# Autodesk Inventor assembly: Assembly1
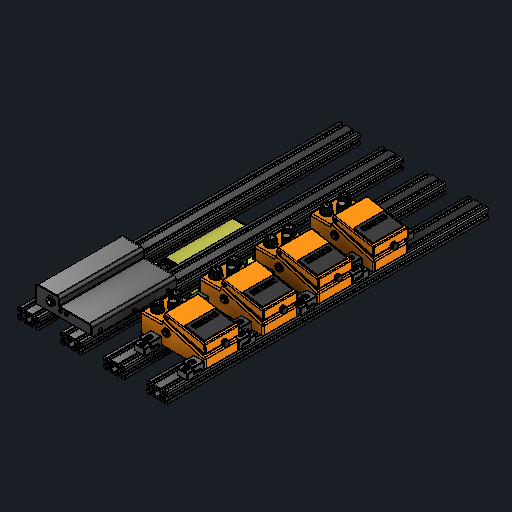
[picture p0: Inventor's stored thumbnail of the model, 512x512]
Saved by Autodesk Inventor 2026.2 (Build 302298000, 298)
## iProperties
Created: 2026-07-17
Part Number: Assembly1
Document SubType Name: Assembly
Designer: JoshuaEah
Author: JoshuaEah
## Documents named in this file (7)
- C:\Users\JoshuaEah\Documents\GitHub\Designed-Trinkets\Guitar\Modular Pedalboard\Assembly1.iam
- C:\Users\JoshuaEah\Documents\GitHub\Designed-Trinkets\Guitar\Modular Pedalboard\Pedals\Boss Pedal\Boss_Assembly.iam
- C:\Users\JoshuaEah\Documents\GitHub\Designed-Trinkets\Guitar\Modular Pedalboard\Fixtures\Fixture Assembly (M4).iam
- C:\Users\JoshuaEah\Documents\GitHub\Designed-Trinkets\Guitar\Modular Pedalboard\Pedals\SuperBlock US\SuperBlock US.iam
- C:\Users\JoshuaEah\Documents\GitHub\Designed-Trinkets\Guitar\Modular Pedalboard\Pedals\Power Supply\VITOOS AD5S LINK.iam
- C:\Users\JoshuaEah\Documents\GitHub\Designed-Trinkets\Guitar\Modular Pedalboard\Hardware\2040x60cm Extrusion.ipt
- 2040x60cm Extrusion.ipt
## Components (26 placed, 5 different names)
1. 2040x60cm Extrusion:5 — Mate:1, Rigid:1, Mate:2, Mate:3, Angle:1, Flush:1, Rigid:2, Mate:6, Mate:8, Planar:1, Flush:4, Flush:5, Planar:6, Planar:7, Mate:18, Mate:19, Mate:29, Mate:30, Planar:9, Flush:6, Planar:11, Mate:38, Mate:40, Planar:15, Planar:16, Flush:7
2. 2040x60cm Extrusion:6 — Rigid:1, Mate:11, Planar:2, Planar:3, Mate:12, Planar:4, Planar:5, Mate:14, Mate:15, Mate:26, Mate:27, Mate:28, Planar:8, Planar:10, Mate:37, Mate:39, Mate:41, Planar:13, Planar:14
3. 2040x60cm Extrusion:7 — Rigid:2, Rigid:3, Mate:31, Mate:32, Planar:12
4. 2040x60cm Extrusion:8 — Rigid:3
5. Boss_Assembly:1 [sub-assembly] — Mate:2, Mate:9, Mate:10, Mate:13, Flush:5, Mate:42
6. Fixture Assembly (M4):1 [sub-assembly] — Mate:3, Angle:1, Flush:1, Mate:10
7. Fixture Assembly (M4):2 [sub-assembly] — Mate:8, Planar:1, Mate:9
8. Fixture Assembly (M4):3 [sub-assembly] — Mate:11, Planar:2, Mate:42
9. Fixture Assembly (M4):4 [sub-assembly] — Planar:3, Mate:12, Mate:13
10. Boss_Assembly:2 [sub-assembly] — Mate:6, Mate:16, Mate:17, Flush:4, Mate:20, Mate:21
11. Fixture Assembly (M4):5 [sub-assembly] — Planar:4, Mate:14, Mate:16
12. Fixture Assembly (M4):6 [sub-assembly] — Planar:5, Mate:15, Mate:17
13. Fixture Assembly (M4):7 [sub-assembly] — Planar:6, Mate:18, Mate:20
14. Fixture Assembly (M4):8 [sub-assembly] — Planar:7, Mate:19, Mate:21
15. Boss_Assembly:3 [sub-assembly] — Mate:25, Mate:27, Flush:6
16. Fixture Assembly (M4):9 [sub-assembly] — Mate:29, Planar:11
17. Fixture Assembly (M4):10 [sub-assembly] — Mate:30, Planar:9
18. Fixture Assembly (M4):11 [sub-assembly] — Mate:25, Mate:26, Planar:8
19. Fixture Assembly (M4):12 [sub-assembly] — Mate:28, Planar:10
20. Boss_Assembly:4 [sub-assembly] — Mate:41, Flush:7
21. Fixture Assembly (M4):13 [sub-assembly] — Mate:37, Planar:13
22. Fixture Assembly (M4):14 [sub-assembly] — Mate:39, Planar:14
23. Fixture Assembly (M4):15 [sub-assembly] — Mate:38, Planar:16
24. Fixture Assembly (M4):16 [sub-assembly] — Mate:40, Planar:15
25. SuperBlock US:1 [sub-assembly] — Mate:31
26. VITOOS AD5S LINK:1 [sub-assembly] — Mate:32, Planar:12
## Relationships (64: Mate 39, PlanarJoint 16, Flush 5, WeldJoint 3, Angle 1)
- Mate:1: 2040x60cm Extrusion:5
- Rigid:1 [WeldJoint] (40 mm): 2040x60cm Extrusion:5 ↔ 2040x60cm Extrusion:6
- Mate:2: 2040x60cm Extrusion:5 ↔ Boss_Assembly:1
- Mate:3: 2040x60cm Extrusion:5 ↔ Fixture Assembly (M4):1
- Angle:1 (0 deg): 2040x60cm Extrusion:5 ↔ Fixture Assembly (M4):1
- Flush:1: 2040x60cm Extrusion:5 ↔ Fixture Assembly (M4):1
- Rigid:2 [WeldJoint] (40 mm): 2040x60cm Extrusion:5 ↔ 2040x60cm Extrusion:7
- Mate:6: 2040x60cm Extrusion:5 ↔ Boss_Assembly:2
- Mate:8: 2040x60cm Extrusion:5 ↔ Fixture Assembly (M4):2
- Planar:1: 2040x60cm Extrusion:5 ↔ Fixture Assembly (M4):2
- Mate:9: Boss_Assembly:1 ↔ Fixture Assembly (M4):2
- Mate:10: Boss_Assembly:1 ↔ Fixture Assembly (M4):1
- Mate:11: 2040x60cm Extrusion:6 ↔ Fixture Assembly (M4):3
- Planar:2: 2040x60cm Extrusion:6 ↔ Fixture Assembly (M4):3
- Planar:3: 2040x60cm Extrusion:6 ↔ Fixture Assembly (M4):4
- Mate:12: 2040x60cm Extrusion:6 ↔ Fixture Assembly (M4):4
- Mate:13: Boss_Assembly:1 ↔ Fixture Assembly (M4):4
- Planar:4: 2040x60cm Extrusion:6 ↔ Fixture Assembly (M4):5
- Planar:5: 2040x60cm Extrusion:6 ↔ Fixture Assembly (M4):6
- Mate:14: 2040x60cm Extrusion:6 ↔ Fixture Assembly (M4):5
- Mate:15: 2040x60cm Extrusion:6 ↔ Fixture Assembly (M4):6
- Mate:16: Boss_Assembly:2 ↔ Fixture Assembly (M4):5
- Mate:17: Boss_Assembly:2 ↔ Fixture Assembly (M4):6
- Flush:4: 2040x60cm Extrusion:5 ↔ Boss_Assembly:2
- Flush:5: 2040x60cm Extrusion:5 ↔ Boss_Assembly:1
- Planar:6: 2040x60cm Extrusion:5 ↔ Fixture Assembly (M4):7
- Planar:7: 2040x60cm Extrusion:5 ↔ Fixture Assembly (M4):8
- Mate:18: 2040x60cm Extrusion:5 ↔ Fixture Assembly (M4):7
- Mate:19: 2040x60cm Extrusion:5 ↔ Fixture Assembly (M4):8
- Mate:20: Boss_Assembly:2 ↔ Fixture Assembly (M4):7
- Mate:21: Boss_Assembly:2 ↔ Fixture Assembly (M4):8
- [Mate]: Boss_Assembly:3 ↔ Fixture Assembly (M4):10
- [Mate]: Boss_Assembly:3 ↔ Fixture Assembly (M4):9
- [Mate]: Boss_Assembly:3 ↔ Fixture Assembly (M4):12
- Mate:25: Boss_Assembly:3 ↔ Fixture Assembly (M4):11
- Mate:26: 2040x60cm Extrusion:6 ↔ Fixture Assembly (M4):11
- Mate:27: 2040x60cm Extrusion:6 ↔ Boss_Assembly:3
- Mate:28: 2040x60cm Extrusion:6 ↔ Fixture Assembly (M4):12
- Mate:29: 2040x60cm Extrusion:5 ↔ Fixture Assembly (M4):9
- Mate:30: 2040x60cm Extrusion:5 ↔ Fixture Assembly (M4):10
- Planar:8: 2040x60cm Extrusion:6 ↔ Fixture Assembly (M4):11
- Planar:9: 2040x60cm Extrusion:5 ↔ Fixture Assembly (M4):10
- Planar:10: 2040x60cm Extrusion:6 ↔ Fixture Assembly (M4):12
- Flush:6: 2040x60cm Extrusion:5 ↔ Boss_Assembly:3
- Planar:11: 2040x60cm Extrusion:5 ↔ Fixture Assembly (M4):9
- Rigid:3 [WeldJoint] (40 mm): 2040x60cm Extrusion:7 ↔ 2040x60cm Extrusion:8
- Mate:31: 2040x60cm Extrusion:7 ↔ SuperBlock US:1
- Mate:32: 2040x60cm Extrusion:7 ↔ VITOOS AD5S LINK:1
- Planar:12: 2040x60cm Extrusion:7 ↔ VITOOS AD5S LINK:1
- [Mate]: Boss_Assembly:4 ↔ Fixture Assembly (M4):13
- [Mate]: Boss_Assembly:4 ↔ Fixture Assembly (M4):14
- [Mate]: Boss_Assembly:4 ↔ Fixture Assembly (M4):15
- [Mate]: Boss_Assembly:4 ↔ Fixture Assembly (M4):16
- Mate:37: 2040x60cm Extrusion:6 ↔ Fixture Assembly (M4):13
- Mate:38: 2040x60cm Extrusion:5 ↔ Fixture Assembly (M4):15
- Mate:39: 2040x60cm Extrusion:6 ↔ Fixture Assembly (M4):14
- Mate:40: 2040x60cm Extrusion:5 ↔ Fixture Assembly (M4):16
- Mate:41: 2040x60cm Extrusion:6 ↔ Boss_Assembly:4
- Planar:13: 2040x60cm Extrusion:6 ↔ Fixture Assembly (M4):13
- Planar:14: 2040x60cm Extrusion:6 ↔ Fixture Assembly (M4):14
- Planar:15: 2040x60cm Extrusion:5 ↔ Fixture Assembly (M4):16
- Planar:16: 2040x60cm Extrusion:5 ↔ Fixture Assembly (M4):15
- Flush:7: 2040x60cm Extrusion:5 ↔ Boss_Assembly:4
- Mate:42: Boss_Assembly:1 ↔ Fixture Assembly (M4):3
## Named parameters: d50_d28 = 0 mm, d51_d29 = 0 mm, d52_d35 = 0 mm, d71_d41 = 0 mm, d72_d48 = 0 mm, d73_d49 = 0 mm, d74_d40 = 0 mm
